# Autodesk Inventor assembly: Passthrough Assembly
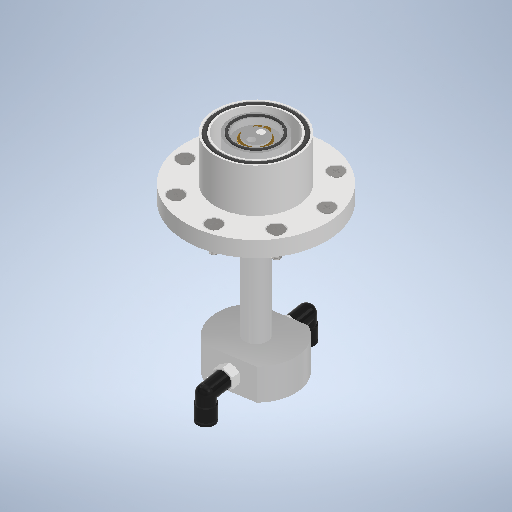
[picture p0: Inventor's stored thumbnail of the model, 512x512]
Saved by Autodesk Inventor 2025 (Build 290162000, 162)
## iProperties
Created: 2024-04-16
Part Number: Passthrough Assembly
Document SubType Name: Assembly
Designer: cfang
Author: cfang
## Documents named in this file (12)
- C:\Users\cfang\Desktop\nebraska-silicon-lab\Hardware\General Gantry\Vacuum Passthrough\Passthrough Assembly.iam
- C:\Users\cfang\Desktop\nebraska-silicon-lab\Hardware\General Gantry\Vacuum Passthrough\Passthrough Spindle.ipt
- C:\Users\cfang\Desktop\nebraska-silicon-lab\Hardware\General Gantry\Vacuum Passthrough\5111K594_Push-to-Connect Tube Fitting for Air and Water\5111K594_Push-to-Connect Tube Fitting for Air and Water.ipt
- C:\Users\cfang\Desktop\nebraska-silicon-lab\Hardware\General Gantry\Vacuum Passthrough\Passthrough Base.ipt
- C:\Users\cfang\Desktop\nebraska-silicon-lab\Hardware\General Gantry\Gantry Tool Holder - Phase II\9396K153 Silicone O-Ring .ipt
- C:\Users\cfang\Desktop\nebraska-silicon-lab\Hardware\General Gantry\Vacuum Passthrough\Passthrough Base Insert.ipt
- C:\Users\cfang\Desktop\nebraska-silicon-lab\Hardware\General Gantry\Vacuum Passthrough\90967A180_External Retaining Ring\90967A180_External Retaining Ring.ipt
- C:\Users\cfang\Desktop\nebraska-silicon-lab\Hardware\General Gantry\Vacuum Passthrough\Aerotech-ADRS150-TT1\Aerotech-ADRS150-TT1.ipt
- C:\Users\cfang\Desktop\nebraska-silicon-lab\Hardware\General Gantry\Vacuum Passthrough\9262K313_Oil-Resistant Buna-N O-Ring\9262K313_Oil-Resistant Buna-N O-Ring.ipt
- C:\Users\cfang\Desktop\nebraska-silicon-lab\Hardware\General Gantry\Vacuum Passthrough\Passthrough Spindle Plug.ipt
- C:\Users\cfang\Desktop\nebraska-silicon-lab\Hardware\General Gantry\Vacuum Passthrough\92010A326_Passivated 18-8 Stainless Steel Phillips Flat Head Screw\92010A326_Passivated 18-8 Stainless Steel Phillips Flat .ipt
- C:\Users\cfang\Desktop\nebraska-silicon-lab\Hardware\General Gantry\Vacuum Passthrough\9262K159_Oil-Resistant Buna-N O-Ring\9262K159_Oil-Resistant Buna-N O-Ring.ipt
## Components (20 placed, 11 different names)
1. Passthrough Spindle:1 — Insert:1, Insert:2, Insert:7, Insert:8, Insert:11, Angle:1, Angle:2, Insert:20, Insert:21
2. 5111K594_Push-to-Connect Tube Fitting for Air and Water:1 — Insert:1, Angle:2
3. 5111K594_Push-to-Connect Tube Fitting for Air and Water:2 — Insert:2, Angle:1
4. Passthrough Base:1 — Insert:3, Insert:4, Mate:1, Insert:9, Insert:12, Insert:13, Insert:14, Insert:15, Insert:16, Insert:17, Insert:18, Insert:19
5. 9396K153 Silicone O-Ring :1 — Insert:3
6. Passthrough Base Insert:1 — Insert:4, Insert:7, Insert:10
7. 90967A180_External Retaining Ring:1 — Insert:8
8. Aerotech-ADRS150-TT1:1 — Mate:1, Insert:9
9. 9262K313_Oil-Resistant Buna-N O-Ring:1 — Insert:10
10. Passthrough Spindle Plug:1 — Insert:11
11. 92010A326_Passivated 18-8 Stainless Steel Phillips Flat :1 — Insert:12
12. 92010A326_Passivated 18-8 Stainless Steel Phillips Flat :2 — Insert:13
13. 92010A326_Passivated 18-8 Stainless Steel Phillips Flat :3 — Insert:14
14. 92010A326_Passivated 18-8 Stainless Steel Phillips Flat :4 — Insert:15
15. 92010A326_Passivated 18-8 Stainless Steel Phillips Flat :5 — Insert:16
16. 92010A326_Passivated 18-8 Stainless Steel Phillips Flat :6 — Insert:17
17. 92010A326_Passivated 18-8 Stainless Steel Phillips Flat :7 — Insert:18
18. 92010A326_Passivated 18-8 Stainless Steel Phillips Flat :8 — Insert:19
19. 9262K159_Oil-Resistant Buna-N O-Ring:1 — Insert:21
20. 9262K159_Oil-Resistant Buna-N O-Ring:2 — Insert:20
## Relationships (22: Insert 19, Angle 2, Mate 1)
- Insert:1: Passthrough Spindle:1 ↔ 5111K594_Push-to-Connect Tube Fitting for Air and Water:1
- Insert:2: Passthrough Spindle:1 ↔ 5111K594_Push-to-Connect Tube Fitting for Air and Water:2
- Insert:3: Passthrough Base:1 ↔ 9396K153 Silicone O-Ring :1
- Insert:4: Passthrough Base:1 ↔ Passthrough Base Insert:1
- Insert:7 (1.75 mm): Passthrough Spindle:1 ↔ Passthrough Base Insert:1
- Insert:8: Passthrough Spindle:1 ↔ 90967A180_External Retaining Ring:1
- Mate:1: Passthrough Base:1 ↔ Aerotech-ADRS150-TT1:1
- Insert:9: Passthrough Base:1 ↔ Aerotech-ADRS150-TT1:1
- Insert:10: Passthrough Base Insert:1 ↔ 9262K313_Oil-Resistant Buna-N O-Ring:1
- Insert:11: Passthrough Spindle:1 ↔ Passthrough Spindle Plug:1
- Insert:12: Passthrough Base:1 ↔ 92010A326_Passivated 18-8 Stainless Steel Phillips Flat :1
- Insert:13: Passthrough Base:1 ↔ 92010A326_Passivated 18-8 Stainless Steel Phillips Flat :2
- Insert:14: Passthrough Base:1 ↔ 92010A326_Passivated 18-8 Stainless Steel Phillips Flat :3
- Insert:15: Passthrough Base:1 ↔ 92010A326_Passivated 18-8 Stainless Steel Phillips Flat :4
- Insert:16: Passthrough Base:1 ↔ 92010A326_Passivated 18-8 Stainless Steel Phillips Flat :5
- Insert:17: Passthrough Base:1 ↔ 92010A326_Passivated 18-8 Stainless Steel Phillips Flat :6
- Insert:18: Passthrough Base:1 ↔ 92010A326_Passivated 18-8 Stainless Steel Phillips Flat :7
- Insert:19: Passthrough Base:1 ↔ 92010A326_Passivated 18-8 Stainless Steel Phillips Flat :8
- Angle:1 (0 deg): Passthrough Spindle:1 ↔ 5111K594_Push-to-Connect Tube Fitting for Air and Water:2
- Angle:2 (0 deg): Passthrough Spindle:1 ↔ 5111K594_Push-to-Connect Tube Fitting for Air and Water:1
- Insert:20 (-0.5 mm): Passthrough Spindle:1 ↔ 9262K159_Oil-Resistant Buna-N O-Ring:2
- Insert:21 (0.5 mm): Passthrough Spindle:1 ↔ 9262K159_Oil-Resistant Buna-N O-Ring:1
